# Autodesk Inventor assembly: FinalAssemblySimplified
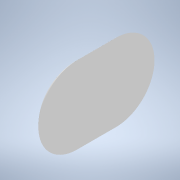
[picture p0: Inventor's stored thumbnail of the model, 180x180]
Saved by Autodesk Inventor 2022 (Build 260153000, 153)
## iProperties
Created: 2022-04-26
Part Number: FinalAssemblySimplified
Document SubType Name: Assembly
Designer: Bruger
Author: Bruger
## Documents named in this file (3)
- C:\Users\Bruger\Desktop\SDU\Civilingeniør\2. Semester\Project in Advanced Robotics\Git\FinalAssemblySimplified.iam
- C:\Users\Bruger\Desktop\SDU\Civilingeniør\2. Semester\Project in Advanced Robotics\Git\3DPrintShapeCornerSimplified.ipt
- C:\Users\Bruger\Desktop\SDU\Civilingeniør\2. Semester\Project in Advanced Robotics\Git\3DPrintShapeStraightEdgeSimplified.ipt
## Components (6 placed, 2 different names)
1. 3DPrintShapeCornerSimplified:1 — Rigid:2
2. 3DPrintShapeCornerSimplified:2 — Rigid:3
3. 3DPrintShapeCornerSimplified:3 — Rigid:4
4. 3DPrintShapeCornerSimplified:4 — Rigid:5
5. 3DPrintShapeStraightEdgeSimplified:1 — Rigid:1, Rigid:2, Rigid:4
6. 3DPrintShapeStraightEdgeSimplified:2 — Rigid:1, Rigid:3, Rigid:5
## Relationships (5: WeldJoint 5)
- Rigid:1 [WeldJoint]: 3DPrintShapeStraightEdgeSimplified:1 ↔ 3DPrintShapeStraightEdgeSimplified:2
- Rigid:2 [WeldJoint]: 3DPrintShapeCornerSimplified:1 ↔ 3DPrintShapeStraightEdgeSimplified:1
- Rigid:3 [WeldJoint]: 3DPrintShapeCornerSimplified:2 ↔ 3DPrintShapeStraightEdgeSimplified:2
- Rigid:4 [WeldJoint]: 3DPrintShapeCornerSimplified:3 ↔ 3DPrintShapeStraightEdgeSimplified:1
- Rigid:5 [WeldJoint]: 3DPrintShapeCornerSimplified:4 ↔ 3DPrintShapeStraightEdgeSimplified:2
